# Autodesk Inventor assembly: Ground_Antenna230mm
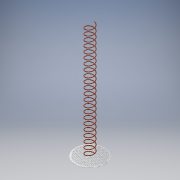
[picture p0: Inventor's stored thumbnail of the model, 180x180]
Saved by Autodesk Inventor 2018 (Build 220112000, 112)
## iProperties
Created: 2018-09-26
Part Number: Ground_Antenna230mm
Document SubType Name: Assembly
Designer: Bradley
Author: Bradley
## Documents named in this file (3)
- C:\Users\Bradley\Documents\CougsInSpace\CougSat1-Hardware\CougSat1-GroundStation\CADModel\Native\Ground_Antenna230mm.iam
- C:\Users\Bradley\Documents\CougsInSpace\CougSat1-Hardware\CougSat1-GroundStation\CADModel\Native\Ground_Antenna230mm_Reflector.ipt
- C:\Users\Bradley\Documents\CougsInSpace\CougSat1-Hardware\CougSat1-GroundStation\CADModel\Native\Ground_Antenna230mm_Helix.ipt
## Components (2 placed, 2 different names)
1. Ground_Antenna230mm_Reflector:1 — Flush:1
2. Ground_Antenna230mm_Helix:1 — Mate:1, Flush:1
## Relationships (2: Mate 1, Flush 1)
- Mate:1: Ground_Antenna230mm_Helix:1
- Flush:1 (2.2 mm): Ground_Antenna230mm_Reflector:1 ↔ Ground_Antenna230mm_Helix:1
